# Autodesk Inventor assembly: Intel_RealSense_Depth_Camera_D435
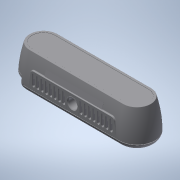
[picture p0: Inventor's stored thumbnail of the model, 180x180]
Saved by Autodesk Inventor 2021.3 (Build 253353000, 353)
## iProperties
Company: INTEL
Created: 2017-10-03
Part Number: Intel_RealSense_Depth_Camera_D435
Material: 一般
Document SubType Name: Assembly
Designer: gisen
Sending System: CREO PARAMETRIC BY PTC INC, 2015380
Preprocessor: CREO PARAMETRIC BY PTC INC, 2015380
Title: D435_RELEASE_ASM_ASM
Author: wkho
Revision Number: 1LAST_VERSION
## Documents named in this file (2)
- C:\Users\gisen\GitProjects\CAD-Data\Devices\RealSenseD435\RealSenseD435.iam
- C:\Users\gisen\GitProjects\CAD-Data\Devices\RealSenseD435\RealSenseD435\000_TA_DS5_DEV_KIT_AWG_RGB_ASM__ASM.iam
## Components (1 placed, 1 different names)
1. 173 [sub-assembly] — メイト:1, メイト:2
## Relationships (2: Mate 2)
- メイト:1 [Mate]: 173
- メイト:2 [Mate]: 173
